# Autodesk Inventor assembly: full_body
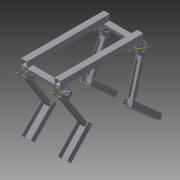
[picture p0: Inventor's stored thumbnail of the model, 180x180]
Saved by Autodesk Inventor 2015 (Build 190159000, 159)
## iProperties
Created: 2014-06-09
Part Number: full_body
Document SubType Name: Assembly
Designer: L
Author: L
## Documents named in this file (3)
- C:\Users\Jaden\Documents\GitHub\SolidModels\stag_v2_01_pre_alpha\full_body.iam
- C:\Users\Jaden\Documents\GitHub\SolidModels\stag_v2_01_pre_alpha\body_frame.ipt
- C:\Users\Jaden\Documents\GitHub\SolidModels\stag_v2_01_pre_alpha\hips_assembly.iam
## Components (4 placed, 2 different names)
1. body_frame:1 — Flush:1, Mate:1, Flush:2
2. body_frame:2 — Flush:3, Flush:4, Mate:2, Flush:5, Mate:3, Flush:6
3. hips_assembly:1 [sub-assembly] — Flush:1, Mate:1, Flush:2, Flush:3, Flush:4, Mate:2
4. hips_assembly:2 [sub-assembly] — Flush:5, Mate:3, Flush:6
## Relationships (9: Flush 6, Mate 3)
- Flush:1: body_frame:1 ↔ hips_assembly:1
- Mate:1: body_frame:1 ↔ hips_assembly:1
- Flush:2: body_frame:1 ↔ hips_assembly:1
- Flush:3: body_frame:2 ↔ hips_assembly:1
- Flush:4: body_frame:2 ↔ hips_assembly:1
- Mate:2: body_frame:2 ↔ hips_assembly:1
- Flush:5: body_frame:2 ↔ hips_assembly:2
- Mate:3: body_frame:2 ↔ hips_assembly:2
- Flush:6: body_frame:2 ↔ hips_assembly:2
